# Autodesk Inventor assembly: 393 Motor CASE ONLY
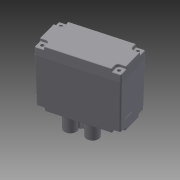
[picture p0: Inventor's stored thumbnail of the model, 180x180]
Saved by Autodesk Inventor 2015 (Build 190159000, 159)
## iProperties
Created: 2016-09-21
Part Number: 393 Motor CASE ONLY
Document SubType Name: Assembly
Designer: L
Author: IFI
Title: 276-2177 Rev1.STEP
Organization: IFI
Description: STEP AP203
Creation Date: 2010-06-25
Sending System: SolidWorks 2009
Preprocessor: SwSTEP 2.0
Author: L
## Documents named in this file (5)
- C:\Users\L\Google Drive\StarStuckProject\Starstruck\VEX Parts\Electronics\Compulsory\393 Motor CASE ONLY.iam
- C:\Users\L\Google Drive\StarStuckProject\Starstruck\Imported Components\393 Motor\276-2177-002 Rev1.ipt
- C:\Users\L\Google Drive\StarStuckProject\Starstruck\Imported Components\393 Motor\276-2177-001 Rev1.ipt
- C:\Users\L\Google Drive\StarStuckProject\Starstruck\Imported Components\393 Motor\276-2177-003 Rev1.ipt
- C:\Users\L\Google Drive\StarStuckProject\Starstruck\Imported Components\393 Motor\276-2177-008 Rev1.ipt
## Components (4 placed, 4 different names)
1. 276-2177-002 Rev1_4 — Mate:1, Mate:2, Mate:3, Mate:4, Tangent:1, Tangent:2, Mate:5
2. 276-2177-001 Rev1_8 — Mate:1, Mate:2, Mate:3
3. 276-2177-003 Rev1_26 — Mate:4, Tangent:1, Tangent:2, Tangent:3
4. 276-2177-008 Rev1:1 — Mate:5, Tangent:3
## Relationships (8: Mate 5, Tangent 3)
- Mate:1: 276-2177-002 Rev1_4 ↔ 276-2177-001 Rev1_8
- Mate:2: 276-2177-002 Rev1_4 ↔ 276-2177-001 Rev1_8
- Mate:3: 276-2177-002 Rev1_4 ↔ 276-2177-001 Rev1_8
- Mate:4: 276-2177-002 Rev1_4 ↔ 276-2177-003 Rev1_26
- Tangent:1 (-1.9 mm): 276-2177-002 Rev1_4 ↔ 276-2177-003 Rev1_26
- Tangent:2 (-1.9 mm): 276-2177-002 Rev1_4 ↔ 276-2177-003 Rev1_26
- Mate:5: 276-2177-002 Rev1_4 ↔ 276-2177-008 Rev1:1
- Tangent:3: 276-2177-003 Rev1_26 ↔ 276-2177-008 Rev1:1
